# Autodesk Inventor assembly: TestAssm
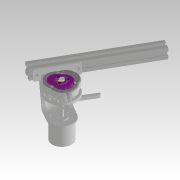
[picture p0: Inventor's stored thumbnail of the model, 180x180]
Saved by Autodesk Inventor 2020 (Build 240168000, 168)
## iProperties
Created: 2021-05-17
Part Number: TestAssm
Document SubType Name: Assembly
Designer: DDeGo
Author: DDeGo
## Documents named in this file (21)
- C:\Users\DDeGo\Documents\Drew\Projects\AirWankelEngine\cad\LiquidPiston V1.5ish\TestAssm.iam
- C:\Users\DDeGo\Documents\Drew\Projects\AirWankelEngine\cad\LiquidPiston V1.5ish\Housing.ipt
- C:\Users\DDeGo\Documents\Drew\Projects\AirWankelEngine\cad\LiquidPiston V1.5ish\Rotor.ipt
- C:\Users\DDeGo\Documents\Drew\Projects\AirWankelEngine\cad\LiquidPiston V1.5ish\CamThing.ipt
- C:\Users\DDeGo\Documents\Drew\Projects\AirWankelEngine\cad\LiquidPiston V1.5ish\TestAssm\Design Accelerator\Spur Gears1.iam
- C:\Users\DDeGo\Documents\Drew\Projects\AirWankelEngine\cad\hardware\6701 bearing.ipt
- C:\Users\DDeGo\Documents\Drew\Projects\AirWankelEngine\cad\LiquidPiston V1.5ish\Head.ipt
- C:\Users\DDeGo\Documents\Drew\Projects\AirWankelEngine\cad\LiquidPiston V1.5ish\ApexSeal.ipt
- C:\Users\DDeGo\Documents\Drew\Projects\AirWankelEngine\cad\hardware\MR85 bearing.ipt
- C:\Users\DDeGo\Documents\Drew\Projects\AirWankelEngine\cad\LiquidPiston V1.5ish\RotorTeeth.ipt
- C:\Users\DDeGo\Documents\Drew\Projects\AirWankelEngine\cad\LiquidPiston V1.5ish\Flywheel.ipt
- C:\Users\DDeGo\Documents\Drew\Projects\AirWankelEngine\cad\hardware\oring_4x2x1.ipt
- C:\Users\DDeGo\Documents\Drew\Projects\AirWankelEngine\cad\hardware\2x22 pin.ipt
- C:\Users\DDeGo\Documents\Drew\Projects\AirWankelEngine\cad\LiquidPiston V1.5ish\ValveThing2.ipt
- C:\Users\DDeGo\Documents\Drew\Projects\AirWankelEngine\cad\LiquidPiston V1.5ish\FlywheelXL.ipt
- C:\Users\DDeGo\Documents\Drew\Projects\AirWankelEngine\cad\LiquidPiston V1.5ish\MotorTestBracket.ipt
- C:\Users\DDeGo\Documents\Drew\Projects\AirWankelEngine\cad\LiquidPiston V1.5ish\2020 Extrusion.ipt
- C:\Users\DDeGo\Documents\Drew\Projects\AirWankelEngine\cad\LiquidPiston V1.5ish\TestLever.ipt
- C:\Users\DDeGo\Documents\Drew\Projects\AirWankelEngine\cad\LiquidPiston V1.5ish\BearingAdapter.ipt
- C:\Users\DDeGo\Documents\Drew\Projects\AirWankelEngine\cad\LiquidPiston V1.5ish\TestEncoderBracket.ipt
- C:\Users\DDeGo\Documents\Drew\Projects\AirWankelEngine\cad\LiquidPiston V1.5ish\TestEncoder.ipt
## Components (25 placed, 20 different names)
1. Housing:1 — Mate:2, Mate:11, Mate:14, Mate:15, Mate:20, Mate:21, Mate:65, Mate:66, Mate:67, Mate:68, Mate:69, Mate:80, Mate:81, Flush:7
2. Rotor:1 — Mate:2, Mate:3, Mate:5, Mate:29, Mate:30, Angle:1, Mate:42, Rotation:1
3. CamThing:1 — Mate:3, Mate:43, Mate:47, Flush:6, Rotation:1
4. Spur Gears:1 [sub-assembly]
5. 6701 bearing:1 — Mate:5, Mate:42, Flush:6
6. ApexSeal:1 — Mate:11, Mate:67
7. ApexSeal:2 — Mate:14, Mate:68
8. ApexSeal:3 — Mate:15, Mate:66
9. MR85 bearing:1 — Mate:20, Mate:21, Mate:32, Mate:33
10. MR85 bearing:2 — Mate:64, Mate:85, Mate:86
11. RotorTeeth:1 — Mate:29, Mate:30, Angle:1
12. Flywheel:1 — Mate:32, Mate:33, Mate:45, Mate:47, Mate:77, Mate:79
13. oring_4x2x1:1 — Flush:2, Flush:3, Mate:71, Tangent:1, Tangent:2
14. oring_4x2x1:2 — Flush:2, Mate:70
15. oring_4x2x1:3 — Flush:3, Mate:72
16. 2x22 pin:1 — Mate:43, Mate:45, Mate:78, Mate:87, Mate:88
17. Head:1 — Mate:64, Mate:65, Mate:69, Mate:70, Mate:71, Mate:72, Tangent:1
18. ValveThing2:1 — Tangent:2
19. FlywheelXL:1 — Mate:77, Mate:78, Mate:79, Mate:83, Mate:84, Mate:93
20. MotorTestBracket:1 — Mate:80, Mate:81, Flush:7, Mate:82, Flush:8, Flush:9
21. 2020 Extrusion:1 — Mate:82, Flush:8, Flush:9, Mate:89, Flush:10
22. TestLever:1 — Mate:83, Mate:84
23. BearingAdapter:1 — Mate:85, Mate:86, Mate:87, Mate:88
24. TestEncoderBracket:1 — Mate:89, Flush:10, Mate:90, Mate:91, Mate:92
25. TestEncoder:1 — Mate:90, Mate:91, Mate:92, Mate:93
## Relationships (53: Mate 42, Flush 7, Tangent 2, Angle 1, RelateRotation 1)
- Mate:2 (0.1 mm): Housing:1 ↔ Rotor:1
- Mate:3: Rotor:1 ↔ CamThing:1
- Mate:5: Rotor:1 ↔ 6701 bearing:1
- Mate:11 (0.1 mm): Housing:1 ↔ ApexSeal:1
- Mate:14 (0.1 mm): Housing:1 ↔ ApexSeal:2
- Mate:15 (0.1 mm): Housing:1 ↔ ApexSeal:3
- Mate:20: Housing:1 ↔ MR85 bearing:1
- Mate:21: Housing:1 ↔ MR85 bearing:1
- Mate:29: Rotor:1 ↔ RotorTeeth:1
- Mate:30: Rotor:1 ↔ RotorTeeth:1
- Angle:1 (0 deg): Rotor:1 ↔ RotorTeeth:1
- Mate:32: MR85 bearing:1 ↔ Flywheel:1
- Mate:33: MR85 bearing:1 ↔ Flywheel:1
- Flush:2: oring_4x2x1:1 ↔ oring_4x2x1:2
- Flush:3: oring_4x2x1:1 ↔ oring_4x2x1:3
- Mate:42: Rotor:1 ↔ 6701 bearing:1
- Mate:43: CamThing:1 ↔ 2x22 pin:1
- Mate:45: Flywheel:1 ↔ 2x22 pin:1
- Mate:47: CamThing:1 ↔ Flywheel:1
- Flush:6: CamThing:1 ↔ 6701 bearing:1
- Mate:64: MR85 bearing:2 ↔ Head:1
- Mate:65: Housing:1 ↔ Head:1
- Mate:66: Housing:1 ↔ ApexSeal:3
- Mate:67: Housing:1 ↔ ApexSeal:1
- Mate:68: Housing:1 ↔ ApexSeal:2
- Mate:69: Housing:1 ↔ Head:1
- Mate:70: oring_4x2x1:2 ↔ Head:1
- Mate:71: oring_4x2x1:1 ↔ Head:1
- Mate:72: oring_4x2x1:3 ↔ Head:1
- Tangent:1: oring_4x2x1:1 ↔ Head:1
- Rotation:1 [RelateRotation] (2 ul): Rotor:1 ↔ CamThing:1
- Mate:77: Flywheel:1 ↔ FlywheelXL:1
- Mate:78: 2x22 pin:1 ↔ FlywheelXL:1
- Mate:79: Flywheel:1 ↔ FlywheelXL:1
- Mate:80: Housing:1 ↔ MotorTestBracket:1
- Mate:81: Housing:1 ↔ MotorTestBracket:1
- Flush:7 (-1 mm): Housing:1 ↔ MotorTestBracket:1
- Mate:82: MotorTestBracket:1 ↔ 2020 Extrusion:1
- Flush:8: MotorTestBracket:1 ↔ 2020 Extrusion:1
- Flush:9 (5 mm): MotorTestBracket:1 ↔ 2020 Extrusion:1
- Mate:83: FlywheelXL:1 ↔ TestLever:1
- Mate:84: FlywheelXL:1 ↔ TestLever:1
- Mate:85: MR85 bearing:2 ↔ BearingAdapter:1
- Mate:86: MR85 bearing:2 ↔ BearingAdapter:1
- Mate:87: 2x22 pin:1 ↔ BearingAdapter:1
- Mate:88: 2x22 pin:1 ↔ BearingAdapter:1
- Tangent:2: oring_4x2x1:1 ↔ ValveThing2:1
- Mate:89: 2020 Extrusion:1 ↔ TestEncoderBracket:1
- Flush:10: 2020 Extrusion:1 ↔ TestEncoderBracket:1
- Mate:90: TestEncoderBracket:1 ↔ TestEncoder:1
- Mate:91: TestEncoderBracket:1 ↔ TestEncoder:1
- Mate:92: TestEncoderBracket:1 ↔ TestEncoder:1
- Mate:93: FlywheelXL:1 ↔ TestEncoder:1
